# Autodesk Inventor assembly: ENSAMBLE GENERAL ACH-40L-2019-V
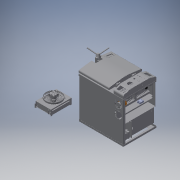
[picture p0: Inventor's stored thumbnail of the model, 180x180]
Saved by Autodesk Inventor 2017 (Build 210142000, 142)
## iProperties
Created: 2020-11-13
Part Number: ENSAMBLE GENERAL ACH-40L-2019-V
Description: STEP AP203
Document SubType Name: Assembly
Designer: USUARIO
Sending System: SolidWorks 2013
Preprocessor: SwSTEP 2.0
Title: ENSAMBLE GENERAL ACH-40L-2019-V.STEP
Revision Number: ANY
## Documents named in this file (22)
- D:\Laboratorio\Autoclave\Autoclave Horizontal\Sin Precamara\2019\Autoclave 40L con Vacio Angelica Castañeda #004588041 OP2019149\Modelo 3D\ENSAMBLE GENERAL ACH-40L-2019-V.iam
- D:\Laboratorio\Autoclave\Autoclave Horizontal\Sin Precamara\2019\Autoclave 40L con Vacio Angelica Castañeda #004588041 OP2019149\Modelo 3D\CUBIERTA FRONTAL ACH-40L-2019-V.ipt
- D:\Laboratorio\Autoclave\Autoclave Horizontal\Sin Precamara\2019\Autoclave 40L con Vacio Angelica Castañeda #004588041 OP2019149\Modelo 3D\BASE MUEBLE ACH-40L-2019-V.ipt
- D:\Laboratorio\Autoclave\Autoclave Horizontal\Sin Precamara\2019\Autoclave 40L con Vacio Angelica Castañeda #004588041 OP2019149\Modelo 3D\ENSAMBLE TANQUE ACH-40L-2019-V.iam
- D:\Laboratorio\Autoclave\Autoclave Horizontal\Sin Precamara\2019\Autoclave 40L con Vacio Angelica Castañeda #004588041 OP2019149\Modelo 3D\ENSAMBLE PANEL FRONTAL ACH-40L-2019-V.iam
- D:\Laboratorio\Autoclave\Autoclave Horizontal\Sin Precamara\2019\Autoclave 40L con Vacio Angelica Castañeda #004588041 OP2019149\Modelo 3D\ENSAMBLE PUERTA ACH-40L-2019-V.iam
- D:\Laboratorio\Autoclave\Autoclave Horizontal\Sin Precamara\2019\Autoclave 40L con Vacio Angelica Castañeda #004588041 OP2019149\Modelo 3D\CUBIERTA SUPERIOR ACH-40L-2019-V.ipt
- D:\Laboratorio\Autoclave\Autoclave Horizontal\Sin Precamara\2019\Autoclave 40L con Vacio Angelica Castañeda #004588041 OP2019149\Modelo 3D\CUBIERTA POSTERIOR ACH-40L-2019-V.ipt
- D:\Laboratorio\Autoclave\Autoclave Horizontal\Sin Precamara\2019\Autoclave 40L con Vacio Angelica Castañeda #004588041 OP2019149\Modelo 3D\CAJA CONEXIONES ESPINAS ACH-40L-2019-V.ipt
- D:\Laboratorio\Autoclave\Autoclave Horizontal\Sin Precamara\2019\Autoclave 40L con Vacio Angelica Castañeda #004588041 OP2019149\Modelo 3D\CALDERIN ACH-40L-2019-V.ipt
- D:\Laboratorio\Autoclave\Autoclave Horizontal\Sin Precamara\2019\Autoclave 40L con Vacio Angelica Castañeda #004588041 OP2019149\Modelo 3D\aislante ACH-40L-2019-V.ipt
- D:\Laboratorio\Autoclave\Autoclave Horizontal\Sin Precamara\2019\Autoclave 40L con Vacio Angelica Castañeda #004588041 OP2019149\Modelo 3D\AISLANTE CALDERIN 40L-2019-V.ipt
- D:\Laboratorio\Autoclave\Autoclave Horizontal\Sin Precamara\2019\Autoclave 40L con Vacio Angelica Castañeda #004588041 OP2019149\Modelo 3D\ULKA EX5.ipt
- D:\Laboratorio\Autoclave\Autoclave Horizontal\Sin Precamara\2019\Autoclave 40L con Vacio Angelica Castañeda #004588041 OP2019149\Modelo 3D\BOMBA DE VACIO THOMAS 2107CA20.ipt
- D:\Laboratorio\Autoclave\Autoclave Horizontal\Sin Precamara\2019\Autoclave 40L con Vacio Angelica Castañeda #004588041 OP2019149\Modelo 3D\ENFRIADOR ACH-40L-2019-V.ipt
- D:\Laboratorio\Autoclave\Autoclave Horizontal\Sin Precamara\2019\Autoclave 40L con Vacio Angelica Castañeda #004588041 OP2019149\Modelo 3D\ANGULO LATERAL ACH-40L-2019.ipt
- D:\Laboratorio\Autoclave\Autoclave Horizontal\Sin Precamara\2019\Autoclave 40L con Vacio Angelica Castañeda #004588041 OP2019149\Modelo 3D\REFUERZO INTERIOR ACH-40L-2019.ipt
- D:\Laboratorio\Autoclave\Autoclave Horizontal\Sin Precamara\2019\Autoclave 40L con Vacio Angelica Castañeda #004588041 OP2019149\Modelo 3D\MANIJA AUTOCLAVE.ipt
- D:\Laboratorio\Autoclave\Autoclave Horizontal\Sin Precamara\2019\Autoclave 40L con Vacio Angelica Castañeda #004588041 OP2019149\Modelo 3D\EnsambleCajaElectrica.iam
- D:\Laboratorio\Autoclave\Autoclave Horizontal\Sin Precamara\2020\Autoclave 40L con Vacio Insulab #004588369 OP2020292\Ensamble General\ENSAMBLE RADIADOR ACH-40L-2020-V.iam
- D:\Laboratorio\Autoclave\Autoclave Horizontal\Sin Precamara\2020\Autoclave 40L con Vacio Insulab #004588369 OP2020292\Ensamble General\RESERVORIO ACH-40L-2020-V.ipt
- D:\Laboratorio\Autoclave\Autoclave Horizontal\Sin Precamara\2019\Autoclave 40L con Vacio Angelica Castañeda #004588041 OP2019149\Modelo 3D\CAJA CONEXIONES ACH-40L-2019.ipt
## Components (22 placed, 22 different names)
1. CUBIERTA FRONTAL ACH-40L-2019-V_1 — Mate:2, Mate:19
2. BASE MUEBLE ACH-40L-2019-V_2 — Mate:1, Mate:3, Mate:4, Mate:9, Mate:11
3. ENSAMBLE TANQUE ACH-40L-2019-V_3 [sub-assembly]
4. ENSAMBLE PANEL FRONTAL ACH-40L-2019-V_4 [sub-assembly]
5. ENSAMBLE PUERTA ACH-40L-2019-V_5 [sub-assembly]
6. CUBIERTA SUPERIOR ACH-40L-2019-V_6
7. CUBIERTA POSTERIOR ACH-40L-2019-V_7 — Mate:10, Mate:14, Mate:15, Mate:17
8. CAJA CONEXIONES ESPINAS ACH-40L-2019-V_8 — Mate:14, Mate:15
9. CALDERIN ACH-40L-2019-V_9
10. aislante ACH-40L-2019-V_10
11. AISLANTE CALDERIN 40L-2019-V_11
12. ULKA EX5_12
13. BOMBA DE VACIO THOMAS 2107CA20_13 — Mate:4, Mate:9
14. ENFRIADOR ACH-40L-2019-V_14
15. ANGULO LATERAL ACH-40L-2019_16
16. ANGULO LATERAL ACH-40L-2019_17
17. REFUERZO INTERIOR ACH-40L-2019_18
18. MANIJA AUTOCLAVE_22
19. EnsambleCajaElectrica:1 [sub-assembly] — Mate:1, Mate:2, Mate:3, Mate:18
20. ENSAMBLE RADIADOR ACH-40L-2020-V:1 [sub-assembly] — Mate:17
21. RESERVORIO ACH-40L-2020-V:1 — Mate:10, Mate:11
22. CAJA CONEXIONES ACH-40L-2019:1 — Mate:18, Mate:19
## Relationships (12: Mate 12)
- Mate:1: BASE MUEBLE ACH-40L-2019-V_2 ↔ EnsambleCajaElectrica:1
- Mate:2 (2 mm): CUBIERTA FRONTAL ACH-40L-2019-V_1 ↔ EnsambleCajaElectrica:1
- Mate:3 (2 mm): BASE MUEBLE ACH-40L-2019-V_2 ↔ EnsambleCajaElectrica:1
- Mate:4: BASE MUEBLE ACH-40L-2019-V_2 ↔ BOMBA DE VACIO THOMAS 2107CA20_13
- Mate:9 (10 mm): BASE MUEBLE ACH-40L-2019-V_2 ↔ BOMBA DE VACIO THOMAS 2107CA20_13
- Mate:10 (5 mm): CUBIERTA POSTERIOR ACH-40L-2019-V_7 ↔ RESERVORIO ACH-40L-2020-V:1
- Mate:11 (20 mm): BASE MUEBLE ACH-40L-2019-V_2 ↔ RESERVORIO ACH-40L-2020-V:1
- Mate:14 (30 mm): CUBIERTA POSTERIOR ACH-40L-2019-V_7 ↔ CAJA CONEXIONES ESPINAS ACH-40L-2019-V_8
- Mate:15: CUBIERTA POSTERIOR ACH-40L-2019-V_7 ↔ CAJA CONEXIONES ESPINAS ACH-40L-2019-V_8
- Mate:17 (2 mm): CUBIERTA POSTERIOR ACH-40L-2019-V_7 ↔ ENSAMBLE RADIADOR ACH-40L-2020-V:1
- Mate:18: EnsambleCajaElectrica:1 ↔ CAJA CONEXIONES ACH-40L-2019:1
- Mate:19 (2 mm): CUBIERTA FRONTAL ACH-40L-2019-V_1 ↔ CAJA CONEXIONES ACH-40L-2019:1
